# Autodesk Inventor assembly: Kepler_Vibe
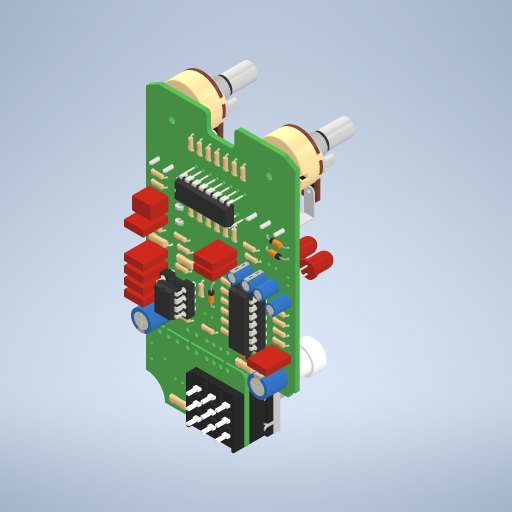
[picture p0: Inventor's stored thumbnail of the model, 512x512]
Saved by Autodesk Inventor 2023 (Build 270158030, 158C)
## iProperties
Created: 2022-11-10
Part Number: Kepler_Vibe
Document SubType Name: Assembly
Designer: Imogen Heard
Author: Imogen Heard
## iProperties of the stored document R_Axial_DIN0411_L9.9mm_D3.6mm_P12.70mm_Horizontal.iam
Created: 2022-11-10
Part Number: R_Axial_DIN0411_L9.9mm_D3.6mm_P12.70mm_Horizontal
Document SubType Name: Assembly
Designer: Imogen Heard
Author: Imogen Heard
## iProperties of the stored document SOLID_5.ipt
Created: 2022-11-10
Part Number: SOLID
Material: Generic
Document SubType Name: Modeling
Designer: Imogen Heard
Density: 1 g/cm^3
Appearance: Default
Author: Imogen Heard
## iProperties of the stored document R_Axial_DIN0411_L9.9mm_D3.6mm_P12.70mm_Horizontal_1.iam
Created: 2022-11-10
Part Number: R_Axial_DIN0411_L9.9mm_D3.6mm_P12.70mm_Horizontal
Document SubType Name: Assembly
Designer: Imogen Heard
Author: Imogen Heard
## iProperties of the stored document DIP-8_W7.62mm.iam
Created: 2022-11-10
Part Number: DIP-8_W7.62mm
Document SubType Name: Assembly
Designer: Imogen Heard
Author: Imogen Heard
## iProperties of the stored document MTS-102.iam
Created: 2022-11-10
Part Number: MTS-102
Document SubType Name: Assembly
Designer: Imogen Heard
Author: Imogen Heard
## iProperties of the stored document SOLID_9.ipt
Created: 2022-11-10
Part Number: SOLID
Material: Generic
Document SubType Name: Modeling
Designer: Imogen Heard
Density: 1 g/cm^3
Appearance: Default
Author: Imogen Heard
## iProperties of the stored document DIP-16_W7.62mm.iam
Created: 2022-11-10
Part Number: DIP-16_W7.62mm
Document SubType Name: Assembly
Designer: Imogen Heard
Author: Imogen Heard
## iProperties of the stored document COMPOUND_1.ipt
Created: 2022-11-10
Part Number: COMPOUND
Material: Generic
Document SubType Name: Modeling
Designer: Imogen Heard
Density: 1 g/cm^3
Appearance: Default
Author: Imogen Heard
## iProperties of the stored document COMPOUND.ipt
Created: 2022-11-10
Part Number: COMPOUND
Material: Generic
Document SubType Name: Modeling
Designer: Imogen Heard
Density: 1 g/cm^3
Appearance: Default
Author: Imogen Heard
## iProperties of the stored document C_Rect_L10.3mm_W7.2mm_P7.50mm_MKS4.iam
Created: 2022-11-10
Part Number: C_Rect_L10.3mm_W7.2mm_P7.50mm_MKS4
Document SubType Name: Assembly
Designer: Imogen Heard
Author: Imogen Heard
## iProperties of the stored document CP_Radial_D12.5mm_P5.00mm.iam
Created: 2022-11-10
Part Number: CP_Radial_D12.5mm_P5.00mm
Document SubType Name: Assembly
Designer: Imogen Heard
Author: Imogen Heard
## iProperties of the stored document DIP-14_W7.62mm.iam
Created: 2022-11-10
Part Number: DIP-14_W7.62mm
Document SubType Name: Assembly
Designer: Imogen Heard
Author: Imogen Heard
## iProperties of the stored document 16mm PCB Pot.iam
Created: 2022-11-10
Part Number: 16mm PCB Pot
Document SubType Name: Assembly
Designer: Imogen Heard
Author: Imogen Heard
## iProperties of the stored document Kepler_Vibe.iam
Company: Kicad
Created: 2022-11-10
Part Number: Kepler_Vibe 1
Description: KiCad electronic assembly
Document SubType Name: Assembly
Designer: Imogen Heard
Authority: Unknown
Sending System: KiCad to STEP converter
Preprocessor: Open CASCADE STEP processor 7.5
Title: Kepler_Vibe.step
Author: Pcbnew
## iProperties of the stored document SOLID_3.ipt
Created: 2022-11-10
Part Number: SOLID
Material: Generic
Document SubType Name: Modeling
Designer: Imogen Heard
Density: 1 g/cm^3
Appearance: Default
Author: Imogen Heard
## iProperties of the stored document Diode 1N4148.iam
Created: 2022-11-10
Part Number: Diode 1N4148
Document SubType Name: Assembly
Designer: Imogen Heard
Author: Imogen Heard
## iProperties of the stored document COMPOUND_2.ipt
Created: 2022-11-10
Part Number: COMPOUND
Material: Generic
Document SubType Name: Modeling
Designer: Imogen Heard
Density: 1 g/cm^3
Appearance: Default
Author: Imogen Heard
## iProperties of the stored document SOLID_7.ipt
Created: 2022-11-10
Part Number: SOLID
Material: Generic
Document SubType Name: Modeling
Designer: Imogen Heard
Density: 1 g/cm^3
Appearance: Default
Author: Imogen Heard
## iProperties of the stored document SOLID_4.ipt
Created: 2022-11-10
Part Number: SOLID
Material: Generic
Document SubType Name: Modeling
Designer: Imogen Heard
Density: 1 g/cm^3
Appearance: Default
Author: Imogen Heard
## iProperties of the stored document SOLID_6.ipt
Created: 2022-11-10
Part Number: SOLID
Material: Generic
Document SubType Name: Modeling
Designer: Imogen Heard
Density: 1 g/cm^3
Appearance: Default
Author: Imogen Heard
## iProperties of the stored document SOLID_11.ipt
Created: 2022-11-10
Part Number: SOLID
Material: Generic
Document SubType Name: Modeling
Designer: Imogen Heard
Density: 1 g/cm^3
Appearance: Default
Author: Imogen Heard
## iProperties of the stored document SOLID_2.ipt
Created: 2022-11-10
Part Number: SOLID
Material: Generic
Document SubType Name: Modeling
Designer: Imogen Heard
Density: 1 g/cm^3
Appearance: Default
Author: Imogen Heard
## iProperties of the stored document SOLID.ipt
Created: 2022-11-10
Part Number: SOLID
Material: Generic
Document SubType Name: Modeling
Designer: Imogen Heard
Density: 1 g/cm^3
Appearance: Default
Author: Imogen Heard
## iProperties of the stored document SOLID_10.ipt
Created: 2022-11-10
Part Number: SOLID
Material: Generic
Document SubType Name: Modeling
Designer: Imogen Heard
Density: 1 g/cm^3
Appearance: Default
Author: Imogen Heard
## iProperties of the stored document _autosave-Tri-Vibe PCB.ipt
Created: 2022-11-10
Part Number: _autosave-Tri-Vibe PCB
Material: Generic
Document SubType Name: Modeling
Designer: Imogen Heard
Density: 1 g/cm^3
Appearance: Default
Author: Imogen Heard
## iProperties of the stored document 3PDT_Footswitch.ipt
Created: 2017-11-16
Part Number: Toggle_Footswitch
Material: Steel
Document SubType Name: Modeling
Designer: Imogen Heard
Density: 7.85 g/cm^3
Appearance: Default
Sending System: Autodesk Translation Framework v6.5.0.72
Preprocessor: ST-DEVELOPER v16.13
Title: /Volumes/BACK UP/3D Shapes/3PDT_footswitch/3PDT_Footswitch.step
Author: mscientistlab
## iProperties of the stored document C_Rect_L7.2mm_W2.5mm_P5.00mm_FKS2_FKP2_MKS2_MKP2.iam
Created: 2022-11-10
Part Number: C_Rect_L7.2mm_W2.5mm_P5.00mm_FKS2_FKP2_MKS2_MKP2
Document SubType Name: Assembly
Designer: Imogen Heard
Author: Imogen Heard
## iProperties of the stored document CP_Radial_D10.0mm_P5.00mm_P7.50mm.iam
Created: 2022-11-10
Part Number: CP_Radial_D10.0mm_P5.00mm_P7.50mm
Document SubType Name: Assembly
Designer: Imogen Heard
Author: Imogen Heard
## iProperties of the stored document DIP-14_W7.62mm_Socket.iam
Created: 2022-11-10
Part Number: DIP-14_W7.62mm_Socket
Document SubType Name: Assembly
Designer: Imogen Heard
Author: Imogen Heard
## iProperties of the stored document LED_D5.0mm.iam
Created: 2022-11-10
Part Number: LED_D5.0mm
Document SubType Name: Assembly
Designer: Imogen Heard
Author: Imogen Heard
## iProperties of the stored document SOLID_1.ipt
Created: 2022-11-10
Part Number: SOLID
Material: Generic
Document SubType Name: Modeling
Designer: Imogen Heard
Density: 1 g/cm^3
Appearance: Default
Author: Imogen Heard
## iProperties of the stored document SOLID_8.ipt
Created: 2022-11-10
Part Number: SOLID
Material: Generic
Document SubType Name: Modeling
Designer: Imogen Heard
Density: 1 g/cm^3
Appearance: Default
Author: Imogen Heard
## iProperties of the stored document DIP-8_W7.62mm_Socket.iam
Created: 2022-11-10
Part Number: DIP-8_W7.62mm_Socket
Document SubType Name: Assembly
Designer: Imogen Heard
Author: Imogen Heard
## Documents named in this file (36)
- C:\Users\dheard\Documents\Inventor\Inventor_Projects\Electronics Projects\Kepler_Vibe.iam
- **C:\Users\dheard\Documents\Inventor\Inventor_Projects\Electronics Projects\Kepler_Vibe.iam*LocalDocs*xAaaaq1caAaaaaaaaAaaaarzxMg*Kepler_Vibe.iam
- **C:\Users\dheard\Documents\Inventor\Inventor_Projects\Electronics Projects\Kepler_Vibe.iam*LocalDocs*xAaaaqpdaAaaaaaaaAaaaa5r3Fh*3PDT_Footswitch.ipt
- **C:\Users\dheard\Documents\Inventor\Inventor_Projects\Electronics Projects\Kepler_Vibe.iam*LocalDocs*xAaaaanaaAaaaaaaaAaaaavhbCc*R_Axial_DIN0411_L9.9mm_D3.6mm_P12.70mm_Horizontal.iam
- **C:\Users\dheard\Documents\Inventor\Inventor_Projects\Electronics Projects\Kepler_Vibe.iam*LocalDocs*xAaaaqlbaAaaaaaaaAaaaa5h5Md*SOLID_10.ipt
- **C:\Users\dheard\Documents\Inventor\Inventor_Projects\Electronics Projects\Kepler_Vibe.iam*LocalDocs*xAaaaafdaAaaaaaaaAaaaqz0wAf*SOLID_5.ipt
- **C:\Users\dheard\Documents\Inventor\Inventor_Projects\Electronics Projects\Kepler_Vibe.iam*LocalDocs*xAaaaa2baAaaaaaaaAaaaq4gdIe*R_Axial_DIN0411_L9.9mm_D3.6mm_P12.70mm_Horizontal_1.iam
- **C:\Users\dheard\Documents\Inventor\Inventor_Projects\Electronics Projects\Kepler_Vibe.iam*LocalDocs*xAaaaqfaaAaaaaaaaAaaaqfdmTc*SOLID_11.ipt
- **C:\Users\dheard\Documents\Inventor\Inventor_Projects\Electronics Projects\Kepler_Vibe.iam*LocalDocs*xAaaaa0caAaaaaaaaAaaaqw4rWf*DIP-8_W7.62mm.iam
- **C:\Users\dheard\Documents\Inventor\Inventor_Projects\Electronics Projects\Kepler_Vibe.iam*LocalDocs*xAaaaq4aaAaaaaaaaAaaaaoxhVb*SOLID_6.ipt
- **C:\Users\dheard\Documents\Inventor\Inventor_Projects\Electronics Projects\Kepler_Vibe.iam*LocalDocs*xAaaaadcaAaaaaaaaAaaaqhndVf*MTS-102.iam
- **C:\Users\dheard\Documents\Inventor\Inventor_Projects\Electronics Projects\Kepler_Vibe.iam*LocalDocs*xAaaaamdaAaaaaaaaAaaaqjhwIb*COMPOUND_1.ipt
- **C:\Users\dheard\Documents\Inventor\Inventor_Projects\Electronics Projects\Kepler_Vibe.iam*LocalDocs*xAaaaambaAaaaaaaaAaaaqgthEf*SOLID_9.ipt
- **C:\Users\dheard\Documents\Inventor\Inventor_Projects\Electronics Projects\Kepler_Vibe.iam*LocalDocs*xAaaaahbaAaaaaaaaAaaaaongDf*DIP-16_W7.62mm.iam
- **C:\Users\dheard\Documents\Inventor\Inventor_Projects\Electronics Projects\Kepler_Vibe.iam*LocalDocs*xAaaaq3daAaaaaaaaAaaaql23Ca*COMPOUND.ipt
- **C:\Users\dheard\Documents\Inventor\Inventor_Projects\Electronics Projects\Kepler_Vibe.iam*LocalDocs*xAaaaawcaAaaaaaaaAaaaahf04c*C_Rect_L10.3mm_W7.2mm_P7.50mm_MKS4.iam
- **C:\Users\dheard\Documents\Inventor\Inventor_Projects\Electronics Projects\Kepler_Vibe.iam*LocalDocs*xAaaaqxdaAaaaaaaaAaaaqaep2b*SOLID_1.ipt
- **C:\Users\dheard\Documents\Inventor\Inventor_Projects\Electronics Projects\Kepler_Vibe.iam*LocalDocs*xAaaaaqcaAaaaaaaaAaaaavxjZb*CP_Radial_D12.5mm_P5.00mm.iam
- **C:\Users\dheard\Documents\Inventor\Inventor_Projects\Electronics Projects\Kepler_Vibe.iam*LocalDocs*xAaaaqacaAaaaaaaaAaaaqrziHe*SOLID_4.ipt
- **C:\Users\dheard\Documents\Inventor\Inventor_Projects\Electronics Projects\Kepler_Vibe.iam*LocalDocs*xAaaaaocaAaaaaaaaAaaaqxb0Rh*DIP-14_W7.62mm.iam
- **C:\Users\dheard\Documents\Inventor\Inventor_Projects\Electronics Projects\Kepler_Vibe.iam*LocalDocs*xAaaaqibaAaaaaaaaAaaaayrdOc*SOLID_7.ipt
- **C:\Users\dheard\Documents\Inventor\Inventor_Projects\Electronics Projects\Kepler_Vibe.iam*LocalDocs*xAaaaavbaAaaaaaaaAaaaa1t1Wa*16mm PCB Pot.iam
- **C:\Users\dheard\Documents\Inventor\Inventor_Projects\Electronics Projects\Kepler_Vibe.iam*LocalDocs*xAaaaqnaaAaaaaaaaAaaaazba3b*COMPOUND_2.ipt
- **C:\Users\dheard\Documents\Inventor\Inventor_Projects\Electronics Projects\Kepler_Vibe.iam*LocalDocs*xAaaaqndaAaaaaaaaAaaaaeptCb*C_Rect_L7.2mm_W2.5mm_P5.00mm_FKS2_FKP2_MKS2_MKP2.iam
- **C:\Users\dheard\Documents\Inventor\Inventor_Projects\Electronics Projects\Kepler_Vibe.iam*LocalDocs*xAaaaqvcaAaaaaaaaAaaaqmkc4f*LED_D5.0mm.iam
- **C:\Users\dheard\Documents\Inventor\Inventor_Projects\Electronics Projects\Kepler_Vibe.iam*LocalDocs*xAaaaq2caAaaaaaaaAaaaqrnvWd*Diode 1N4148.iam
- **C:\Users\dheard\Documents\Inventor\Inventor_Projects\Electronics Projects\Kepler_Vibe.iam*LocalDocs*xAaaaqudaAaaaaaaaAaaaqlpvNd*CP_Radial_D10.0mm_P5.00mm_P7.50mm.iam
- **C:\Users\dheard\Documents\Inventor\Inventor_Projects\Electronics Projects\Kepler_Vibe.iam*LocalDocs*xAaaaqybaAaaaaaaaAaaaaodzIe*DIP-8_W7.62mm_Socket.iam
- **C:\Users\dheard\Documents\Inventor\Inventor_Projects\Electronics Projects\Kepler_Vibe.iam*LocalDocs*xAaaaqwaaAaaaaaaaAaaaqhrf1f*DIP-14_W7.62mm_Socket.iam
- **C:\Users\dheard\Documents\Inventor\Inventor_Projects\Electronics Projects\Kepler_Vibe.iam*LocalDocs*xAaaaqvcaAaaaaaaaAaaaaxcxYg*_autosave-Tri-Vibe PCB.ipt
- **C:\Users\dheard\Documents\Inventor\Inventor_Projects\Electronics Projects\Kepler_Vibe.iam*LocalDocs*xAaaaq0baAaaaaaaaAaaaq401Kh*SOLID_3.ipt
- **C:\Users\dheard\Documents\Inventor\Inventor_Projects\Electronics Projects\Kepler_Vibe.iam*LocalDocs*xAaaaqkcaAaaaaaaaAaaaamdxRc*SOLID_2.ipt
- **C:\Users\dheard\Documents\Inventor\Inventor_Projects\Electronics Projects\Kepler_Vibe.iam*LocalDocs*xAaaaqidaAaaaaaaaAaaaa4osOb*SOLID.ipt
- **C:\Users\dheard\Documents\Inventor\Inventor_Projects\Electronics Projects\Kepler_Vibe.iam*LocalDocs*xAaaaqwcaAaaaaaaaAaaaaku3Lg*SOLID_8.ipt
- C:\Users\dheard\Documents\Inventor\Inventor_Projects\Electronics Projects\Kepler_Vibe.step
- C:\Users\dheard\Documents\0000.KiCad\6.0\3rdparty\000_Immo_3D_models\3pdt-footswitch-1.snapshot.3\3PDT_Footswitch.step
## Components (2 placed, 2 different names)
1. Kepler_Vibe:1 [sub-assembly] — Flush:1
2. 3PDT_Footswitch:2 — Flush:1
## Relationships (1: Flush 1)
- Flush:1: Kepler_Vibe:1 ↔ 3PDT_Footswitch:2
